# Autodesk Inventor assembly: Assembly1
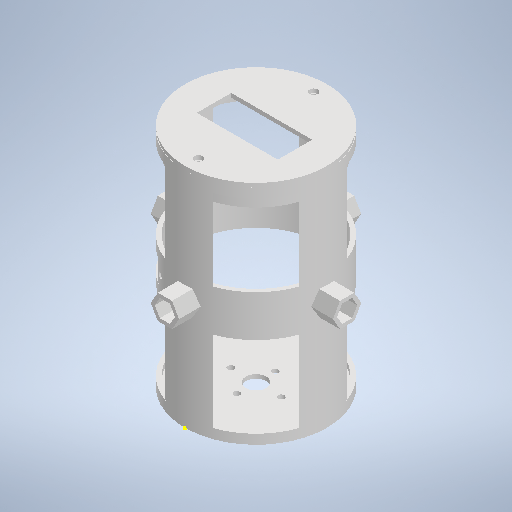
[picture p0: Inventor's stored thumbnail of the model, 512x512]
Saved by Autodesk Inventor 2025.3 (Build 293356000, 356)
## iProperties
Created: 2025-04-18
Part Number: Assembly1
Document SubType Name: Assembly
Designer: Owner
Author: Owner
## Documents named in this file (3)
- D:\JRD301\cad model\Assembly1.iam
- D:\JRD301\cad model\main_body.ipt
- D:\JRD301\cad model\lid2.ipt
## Components (2 placed, 2 different names)
1. main_body:1 — Flush:1, Flush:2
2. lid2:1 — Flush:1, Flush:2
## Relationships (2: Flush 2)
- Flush:1: main_body:1 ↔ lid2:1
- Flush:2: main_body:1 ↔ lid2:1
